# Autodesk Inventor assembly: 出力ピンユニット
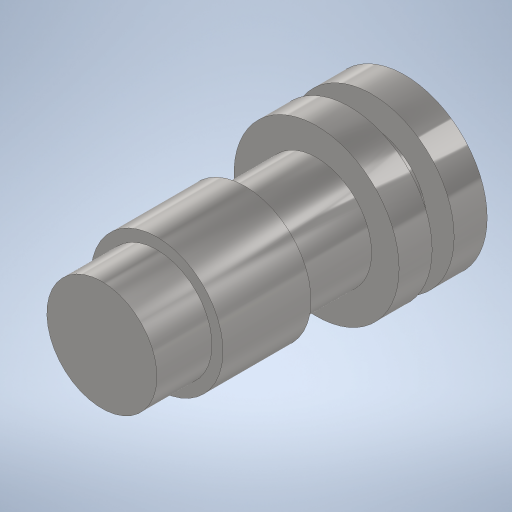
[picture p0: Inventor's stored thumbnail of the model, 512x512]
Saved by Autodesk Inventor 2024 (Build 280153000, 153)
## iProperties
Created: 2023-05-29
Part Number: 出力ピンユニット
Document SubType Name: Assembly
Designer: yuta2
Mass: 11.7389 g
Surface Area: 12.8805 cm^2
Volume: 1.4954 cm^3
Density: 7.85 g/cm^3
Author: yuta2
## Documents named in this file (9)
- C:\Users\yuta2\Documents\Inventor\mokemoke2023\サイクロイド減速機_大型\出力ピンユニット.iam
- C:\Users\yuta2\Documents\Inventor\mokemoke2023\サイクロイド減速機_大型\出力ピン.ipt
- C:\Users\yuta2\Documents\Inventor\mokemoke2023\ベアリング\SMT1510.ipt
- C:\Users\yuta2\Documents\Inventor\mokemoke2023\サイクロイド減速機_大型\出力ピンユニット\AIP\FEA\ecnbbsna8.fins
- C:\Users\yuta2\Documents\Inventor\mokemoke2023\サイクロイド減速機_大型\出力ピンユニット\AIP\FEA\ecnbbsnb4.fsat
- C:\Users\yuta2\Documents\Inventor\mokemoke2023\サイクロイド減速機_大型\出力ピンユニット\AIP\FEA\ecnbbsnb4.ftes
- C:\Users\yuta2\Documents\Inventor\mokemoke2023\サイクロイド減速機_大型\出力ピンユニット\AIP\FEA\ecnbbsnb4.fwiz
- C:\Users\yuta2\Documents\Inventor\mokemoke2023\サイクロイド減速機_大型\出力ピンユニット\AIP\FEA\ecnbbsnc0.fmsh
- C:\Users\yuta2\Documents\Inventor\mokemoke2023\サイクロイド減速機_大型\出力ピンユニット\AIP\FEA\ecnbbsnc1.fres
## Components (3 placed, 2 different names)
1. 出力ピン:1 — 回転:1
2. SMT1510:1 — 回転:2
3. SMT1510:2 — 回転:1, 回転:2
## Relationships (2: RevoluteJoint 2)
- 回転:1 [RevoluteJoint] (0.5 mm): 出力ピン:1 ↔ SMT1510:2
- 回転:2 [RevoluteJoint] (2 mm): SMT1510:1 ↔ SMT1510:2
